# Autodesk Inventor assembly: assembly
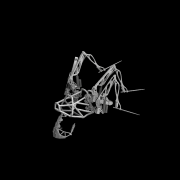
[picture p0: Inventor's stored thumbnail of the model, 180x180]
Saved by Autodesk Inventor 2020 (Build 240168000, 168)
## iProperties
Created: 2020-03-24
Part Number: assembly
Document SubType Name: Assembly
Designer: valer
Author: valer
## Documents named in this file (30)
- C:\Users\valer\Desktop\drummingrobot\src\Robot.iam
- C:\Users\valer\Desktop\drummingrobot\src\Chest.ipt
- C:\Users\valer\Desktop\drummingrobot\src\HeadScaled.ipt
- C:\Users\valer\Desktop\drummingrobot\src\UpperArm.ipt
- C:\Users\valer\Desktop\drummingrobot\src\UpperArmBracket.ipt
- C:\Users\valer\Desktop\drummingrobot\src\external\ShoulderConnectingRod.ipt
- C:\Users\valer\Desktop\drummingrobot\src\Forearm.ipt
- C:\Users\valer\Desktop\drummingrobot\src\external\Drumstick.ipt
- C:\Users\valer\Desktop\drummingrobot\src\external\ForearmShaftCollar.ipt
- C:\Users\valer\Desktop\drummingrobot\src\external\RodEndFixed.ipt
- C:\Users\valer\Desktop\drummingrobot\src\ShoulderBracket.ipt
- C:\Users\valer\Desktop\drummingrobot\src\ChestShoulderBracket.ipt
- C:\Users\valer\Desktop\drummingrobot\src\ChestShoulderBracketMirror.ipt
- C:\Users\valer\Desktop\drummingrobot\src\external\UpperArmActuatorBody.ipt
- C:\Users\valer\Desktop\drummingrobot\src\external\UpperArmActuatorShaft.ipt
- C:\Users\valer\Desktop\drummingrobot\src\external\ForearmActuatorBody.ipt
- C:\Users\valer\Desktop\drummingrobot\src\external\ForearmActuatorShaft.ipt
- C:\Users\valer\Desktop\drummingrobot\src\external\Drums.ipt
- C:\Users\valer\Desktop\drummingrobot\src\ForearmActuatorConnector.ipt
- C:\Users\valer\Desktop\drummingrobot\src\external\ArmRotationServoBody.ipt
- C:\Users\valer\Desktop\drummingrobot\src\external\ArmRotationServoHead.ipt
- C:\Users\valer\Desktop\drummingrobot\src\external\PullSolenoid.ipt
- C:\Users\valer\Desktop\drummingrobot\src\PullSolenoidArmBracket.ipt
- C:\Users\valer\Desktop\drummingrobot\src\UpperShoulderBracket.ipt
- C:\Users\valer\Desktop\drummingrobot\src\UpperArmActuatorBracketAlt.ipt
- C:\Users\valer\Desktop\drummingrobot\src\external\ShockAbsorberDerived.ipt
- C:\Users\valer\Desktop\drummingrobot\src\Spine.ipt
- C:\Users\valer\Desktop\drummingrobot\src\SpineLinkTop.ipt
- C:\Users\valer\Desktop\drummingrobot\src\SpineLinkBottom.ipt
- C:\Users\valer\Desktop\drummingrobot\src\Pelvis.iam
## Components (132 placed, 29 different names)
1. Chest:1 — Angle:6, Mate:117, Mate:118, Mate:119, Mate:120, Mate:121, Mate:122, Mate:130, Mate:131, Mate:132, Mate:133, Mate:134, Mate:157, Angle:12, Mate:425, Mate:426, Mate:427, Mate:428, Mate:429, Mate:430, Mate:431, Mate:432, Mate:433, Mate:434, Mate:435, Mate:436, Angle:18, Mate:568, Mate:571, Angle:23
2. HeadScaled:1 — Angle:6
3. Drumstick:1 — Mate:79, Flush:23, Mate:424
4. ShaftCollar1/2:1 — Mate:79, Mate:290, Mate:291, Flush:23
5. ChestShoulderBracket:1 — Mate:120, Mate:121, Mate:122, Mate:377, Mate:378, Mate:379, Mate:380, Flush:31
6. ChestShoulderBracketMirror:1 — Mate:117, Mate:118, Mate:119, Mate:395, Mate:396, Mate:397, Mate:398
7. ChestShoulderBracket:2 — Mate:130, Mate:131, Mate:157, Mate:160, Mate:162, Mate:213, Mate:214, Flush:28
8. ChestShoulderBracketMirror:2 — Mate:132, Mate:133, Mate:134, Mate:141, Mate:146, Mate:148, Mate:149
9. ChestConnectingRod:5
10. ChestConnectingRod:6
11. RodEnd1/4-1/4-1:9 — Mate:342
12. RodEnd1/4-1/4-1:10 — Mate:148, Mate:149
13. RodEnd1/4-1/4-1:11 — Mate:341
14. RodEnd1/4-1/4-1:12 — Mate:141, Mate:146
15. ChestConnectingRod:7
16. ChestConnectingRod:8
17. RodEnd1/4-1/4-1:13 — Mate:340
18. RodEnd1/4-1/4-1:14 — Mate:162, Mate:214
19. RodEnd1/4-1/4-1:15 — Mate:339
20. RodEnd1/4-1/4-1:16 — Mate:160, Mate:213
21. UpperArmActuatorBody:1 — Mate:182, Mate:183, Mate:423
22. Forearm:1 — Flush:17, Mate:227, Mate:239, Mate:244, Mate:290, Mate:291, Mate:293, Mate:296
23. UpperArmActuatorShaft:2 — Mate:182, Mate:183, Mate:238, Flush:20
24. ForearmActuatorBody:1 — Mate:231, Mate:232, Mate:234, Flush:19
25. Drums:1
26. ForearmActuatorShaft:3 — Flush:17, Mate:231, Mate:232, Mate:241, Mate:243, Angle:10, Mate:246
27. UpperArm:3 — Mate:227, Mate:234, Mate:238, Flush:19, Flush:20, Mate:249, Mate:287
28. ForearmActuatorConnector:1 — Mate:239, Mate:241, Mate:245, Angle:10, Mate:246
29. ForearmActuatorConnector:2 — Mate:243, Mate:244, Mate:245
30. UpperArmBracket:5 — Mate:249, Mate:287, Mate:420, Mate:421, Mate:454
31. ArmRotationServoBody:1 — Mate:258, Mate:259, Angle:12, Mate:384, Mate:386, Mate:387, Mate:388, Mate:402
32. ArmRotationServoHead:1 — Mate:258, Mate:259, Mate:417, Mate:418, Mate:453
33. PullSolenoid:1 — Mate:294, Mate:295, Angle:16, Mate:424
34. PullSolenoidArmBracket:1 — Mate:293, Mate:294, Mate:295, Mate:296, Angle:16
35. Forearm:2 — Mate:343, Mate:347, Mate:352, Mate:353
36. ShaftCollar1/2:2 — Mate:354, Flush:29
37. ShoulderBracket:6 — Mate:332, Mate:333, Flush:28, Mate:339, Mate:340, Mate:403
38. UpperArmActuatorBody:2 — Mate:416
39. UpperArmActuatorShaft:3
40. ForearmActuatorBody:2
41. ForearmActuatorShaft:4 — Mate:349, Mate:350, Mate:351, Angle:13
42. UpperArm:4
43. UpperArmBracket:6 — Mate:413, Mate:414, Mate:415
44. ArmRotationServoBody:2 — Mate:330, Mate:331, Mate:332, Mate:333, Mate:334, Mate:335, Mate:403, Mate:404
45. ShoulderBracket:7 — Mate:334, Mate:335, Mate:341, Mate:342, Mate:404
46. PullSolenoid:2 — Mate:344, Mate:345, Angle:14, Mate:355
47. PullSolenoidArmBracket:2 — Mate:343, Mate:344, Mate:345, Mate:347, Angle:14
48. ArmRotationServoHead:2 — Mate:330, Mate:331, Mate:410, Mate:411, Mate:412
49. ForearmActuatorConnector:3 — Mate:349, Mate:351, Mate:353
50. ForearmActuatorConnector:4 — Mate:350, Mate:352, Angle:13
51. Drumstick:2 — Mate:354, Mate:355, Flush:29
52. UpperShoulderBracket:1 — Mate:384, Flush:31, Mate:388, Mate:389, Mate:390
53. UpperShoulderBracket:2 — Mate:386, Mate:387, Mate:391, Mate:392, Mate:401, Mate:402
54. RodEnd1/4-1/4-1:17 — Mate:382, Mate:389
55. RodEnd1/4-1/4-1:18 — Mate:381, Mate:390, Mate:406
56. RodEnd1/4-1/4-1:19 — Mate:377, Mate:378, Mate:382, Mate:405
57. RodEnd1/4-1/4-1:20 — Mate:379, Mate:380, Mate:381
58. RodEnd1/4-1/4-1:21 — Mate:392, Mate:400, Mate:408
59. RodEnd1/4-1/4-1:22 — Mate:391, Mate:399, Mate:401, Mate:407
60. RodEnd1/4-1/4-1:23 — Mate:395, Mate:398, Mate:399
61. RodEnd1/4-1/4-1:24 — Mate:396, Mate:397, Mate:400, Mate:573
62. ChestConnectingRod:9 — Mate:405
63. ChestConnectingRod:10 — Mate:406
64. ChestConnectingRod:11 — Mate:407
65. ChestConnectingRod:12 — Mate:408
66. UpperArmActuatorBracketAlt:1 — Mate:410, Mate:411, Mate:412, Mate:413, Mate:414, Mate:415, Mate:416
67. UpperArmActuatorBracketAlt:2 — Mate:417, Mate:418, Mate:420, Mate:421, Mate:423, Mate:453, Mate:454
68. ChestShoulderBracket:3 — Mate:428, Mate:429, Mate:430, Mate:437, Mate:438, Mate:439, Mate:440
69. ChestShoulderBracketMirror:3 — Mate:425, Mate:426, Mate:427, Mate:441, Mate:442, Mate:443, Mate:444, Mate:570
70. ChestShoulderBracket:4 — Mate:431, Mate:432, Mate:433, Mate:445, Mate:446, Mate:447, Mate:448
71. ChestShoulderBracketMirror:4 — Mate:434, Mate:435, Mate:436, Mate:449, Mate:451, Mate:452
72. RodEnd1/4-1/4-1:25 — Mate:439, Mate:440
73. RodEnd1/4-1/4-1:26 — Mate:437, Mate:438, Mate:481
74. RodEnd1/4-1/4-1:27 — Mate:442, Mate:444, Mate:480
75. RodEnd1/4-1/4-1:28 — Mate:441, Mate:443, Mate:479
76. RodEnd1/4-1/4-1:29 — Mate:447, Mate:448, Mate:499
77. RodEnd1/4-1/4-1:30 — Mate:445, Mate:446, Mate:498
78. RodEnd1/4-1/4-1:31 — Mate:452, Mate:497
79. RodEnd1/4-1/4-1:32 — Mate:449, Mate:451, Mate:496
80. ArmRotationServoBody:3 — Mate:469
81. ArmRotationServoHead:3 — Mate:509, Mate:510, Mate:511
82. UpperShoulderBracket:3 — Mate:469, Mate:474, Mate:476, Mate:567
83. UpperShoulderBracket:4 — Mate:471
84. ArmRotationServoBody:4 — Mate:482, Mate:483, Mate:484, Mate:485, Mate:486, Mate:487, Angle:18
85. ArmRotationServoHead:4 — Mate:521, Mate:522, Mate:523
86. RodEnd1/4-1/4-1:33 — Mate:471, Mate:479
87. RodEnd1/4-1/4-1:34 — Mate:480
88. RodEnd1/4-1/4-1:35 — Mate:481
89. RodEnd1/4-1/4-1:36 — Mate:474, Mate:476
90. RodEnd1/4-1/4-1:37 — Mate:492, Mate:494, Mate:498
91. RodEnd1/4-1/4-1:38 — Mate:493, Mate:495, Mate:499
92. RodEnd1/4-1/4-1:39 — Mate:489, Mate:491, Mate:497
93. RodEnd1/4-1/4-1:40 — Mate:496
94. ShoulderBracket:8 — Mate:482, Mate:483, Mate:484, Mate:489, Mate:491
95. ShoulderBracket:9 — Mate:485, Mate:486, Mate:487, Mate:492, Mate:493, Mate:494, Mate:495, Mate:566
96. UpperArmActuatorBody:3
97. UpperArmActuatorShaft:4
98. UpperArm:5 — Mate:558, Mate:559, Mate:560
99. UpperArmBracket:7
100. UpperArmActuatorBracketAlt:3 — Mate:509, Mate:510, Mate:511
101. UpperArmActuatorBody:4
102. UpperArmActuatorShaft:5
103. UpperArm:6 — Mate:561, Mate:562, Mate:563
104. UpperArmBracket:8
105. UpperArmActuatorBracketAlt:4 — Mate:521, Mate:522, Mate:523
106. Forearm:3 — Mate:558, Mate:559
107. Drumstick:3 — Mate:556
108. ShaftCollar1/2:3 — Mate:556
109. ForearmActuatorBody:3 — Mate:560
110. ForearmActuatorShaft:5
111. ForearmActuatorConnector:5
112. ForearmActuatorConnector:6
113. PullSolenoid:3
114. PullSolenoidArmBracket:3
115. Forearm:4 — Mate:561, Mate:562
116. Drumstick:4 — Mate:557, Mate:564
117. ShaftCollar1/2:4 — Mate:557
118. ForearmActuatorBody:4 — Mate:563
119. ForearmActuatorShaft:6
120. ForearmActuatorConnector:7
121. ForearmActuatorConnector:8
122. PullSolenoid:4 — Mate:564
123. PullSolenoidArmBracket:4
124. ShockAbsorberDerived:1 — Mate:566, Mate:570
125. ShockAbsorberDerived:2 — Mate:567, Mate:568
126. ShockAbsorberDerived:3 — Mate:573
127. ShockAbsorberDerived:4 — Mate:571
128. ShockAbsorberDerived:5 — Mate:585, Mate:586
129. Spine:1 — Mate:574, Mate:575, Mate:576, Mate:579, Mate:580, Mate:581, Mate:582, Mate:583, Mate:584, Angle:23
130. SpineLinkTop:1 — Mate:574, Mate:575, Mate:576
131. SpineLinkBottom:1 — Mate:579, Mate:580, Mate:581
132. Pelvis:1 [sub-assembly] — Mate:582, Mate:583, Mate:584, Mate:585, Mate:586
## Relationships (294: Mate 266, Flush 16, Angle 12)
- Angle:6 (0 deg): Chest:1 ↔ HeadScaled:1
- Mate:79: Drumstick:1 ↔ ShaftCollar1/2:1
- Mate:117: Chest:1 ↔ ChestShoulderBracketMirror:1
- Mate:118: Chest:1 ↔ ChestShoulderBracketMirror:1
- Mate:119: Chest:1 ↔ ChestShoulderBracketMirror:1
- Mate:120: Chest:1 ↔ ChestShoulderBracket:1
- Mate:121: Chest:1 ↔ ChestShoulderBracket:1
- Mate:122: Chest:1 ↔ ChestShoulderBracket:1
- Mate:130: Chest:1 ↔ ChestShoulderBracket:2
- Mate:131: Chest:1 ↔ ChestShoulderBracket:2
- Mate:132: Chest:1 ↔ ChestShoulderBracketMirror:2
- Mate:133: Chest:1 ↔ ChestShoulderBracketMirror:2
- Mate:134: Chest:1 ↔ ChestShoulderBracketMirror:2
- [Mate]: ChestConnectingRod:6 ↔ RodEnd1/4-1/4-1:9
- [Mate]: ChestConnectingRod:6 ↔ RodEnd1/4-1/4-1:10
- [Mate]: ChestConnectingRod:5 ↔ RodEnd1/4-1/4-1:11
- [Mate]: ChestConnectingRod:5 ↔ RodEnd1/4-1/4-1:12
- [Mate] (-25.4 mm): ChestConnectingRod:6 ↔ RodEnd1/4-1/4-1:10
- [Mate] (-25.4 mm): ChestConnectingRod:5 ↔ RodEnd1/4-1/4-1:12
- Mate:141: ChestShoulderBracketMirror:2 ↔ RodEnd1/4-1/4-1:12
- Mate:146: ChestShoulderBracketMirror:2 ↔ RodEnd1/4-1/4-1:12
- Mate:148: ChestShoulderBracketMirror:2 ↔ RodEnd1/4-1/4-1:10
- Mate:149: ChestShoulderBracketMirror:2 ↔ RodEnd1/4-1/4-1:10
- [Mate]: ChestConnectingRod:8 ↔ RodEnd1/4-1/4-1:13
- [Mate]: ChestConnectingRod:8 ↔ RodEnd1/4-1/4-1:14
- [Mate]: ChestConnectingRod:7 ↔ RodEnd1/4-1/4-1:15
- [Mate]: ChestConnectingRod:7 ↔ RodEnd1/4-1/4-1:16
- [Mate] (-25.4 mm): ChestConnectingRod:8 ↔ RodEnd1/4-1/4-1:14
- [Mate] (-25.4 mm): ChestConnectingRod:7 ↔ RodEnd1/4-1/4-1:16
- Mate:157: Chest:1 ↔ ChestShoulderBracket:2
- Mate:160: ChestShoulderBracket:2 ↔ RodEnd1/4-1/4-1:16
- Mate:162: ChestShoulderBracket:2 ↔ RodEnd1/4-1/4-1:14
- Mate:182: UpperArmActuatorBody:1 ↔ UpperArmActuatorShaft:2
- Mate:183: UpperArmActuatorBody:1 ↔ UpperArmActuatorShaft:2
- Mate:213: ChestShoulderBracket:2 ↔ RodEnd1/4-1/4-1:16
- Mate:214: ChestShoulderBracket:2 ↔ RodEnd1/4-1/4-1:14
- Flush:17: Forearm:1 ↔ ForearmActuatorShaft:3
- Mate:227: Forearm:1 ↔ UpperArm:3
- Mate:231: ForearmActuatorBody:1 ↔ ForearmActuatorShaft:3
- Mate:232: ForearmActuatorBody:1 ↔ ForearmActuatorShaft:3
- Mate:234: ForearmActuatorBody:1 ↔ UpperArm:3
- Mate:238: UpperArmActuatorShaft:2 ↔ UpperArm:3
- Flush:19: ForearmActuatorBody:1 ↔ UpperArm:3
- Flush:20: UpperArmActuatorShaft:2 ↔ UpperArm:3
- Mate:239: Forearm:1 ↔ ForearmActuatorConnector:1
- Mate:241: ForearmActuatorShaft:3 ↔ ForearmActuatorConnector:1
- Mate:243: ForearmActuatorShaft:3 ↔ ForearmActuatorConnector:2
- Mate:244: Forearm:1 ↔ ForearmActuatorConnector:2
- Mate:245: ForearmActuatorConnector:1 ↔ ForearmActuatorConnector:2
- Angle:10 (-180 deg): ForearmActuatorShaft:3 ↔ ForearmActuatorConnector:1
- Mate:246: ForearmActuatorShaft:3 ↔ ForearmActuatorConnector:1
- Mate:249: UpperArm:3 ↔ UpperArmBracket:5
- Mate:258: ArmRotationServoBody:1 ↔ ArmRotationServoHead:1
- Mate:259: ArmRotationServoBody:1 ↔ ArmRotationServoHead:1
- Angle:12 (0 deg): Chest:1 ↔ ArmRotationServoBody:1
- Mate:287: UpperArm:3 ↔ UpperArmBracket:5
- Mate:290: ShaftCollar1/2:1 ↔ Forearm:1
- Mate:291 (8.4667 mm): ShaftCollar1/2:1 ↔ Forearm:1
- Mate:293: Forearm:1 ↔ PullSolenoidArmBracket:1
- Mate:294: PullSolenoid:1 ↔ PullSolenoidArmBracket:1
- Mate:295: PullSolenoid:1 ↔ PullSolenoidArmBracket:1
- Mate:296: Forearm:1 ↔ PullSolenoidArmBracket:1
- Flush:23 (302.5394 mm): Drumstick:1 ↔ ShaftCollar1/2:1
- [Mate]: UpperArmActuatorBody:2 ↔ UpperArmActuatorShaft:3
- [Mate]: UpperArmActuatorBody:2 ↔ UpperArmActuatorShaft:3
- [Flush]: Forearm:2 ↔ ForearmActuatorShaft:4
- [Mate]: Forearm:2 ↔ UpperArm:4
- [Mate]: ForearmActuatorBody:2 ↔ ForearmActuatorShaft:4
- [Mate]: ForearmActuatorBody:2 ↔ ForearmActuatorShaft:4
- [Mate]: ForearmActuatorBody:2 ↔ UpperArm:4
- [Mate]: UpperArmActuatorShaft:3 ↔ UpperArm:4
- [Flush]: ForearmActuatorBody:2 ↔ UpperArm:4
- [Flush]: UpperArmActuatorShaft:3 ↔ UpperArm:4
- [Mate]: UpperArm:4 ↔ UpperArmBracket:6
- [Mate]: UpperArm:4 ↔ UpperArmBracket:6
- [Mate]: Forearm:2 ↔ ShaftCollar1/2:2
- [Mate] (8.4667 mm): Forearm:2 ↔ ShaftCollar1/2:2
- Mate:330: ArmRotationServoBody:2 ↔ ArmRotationServoHead:2
- Mate:331: ArmRotationServoBody:2 ↔ ArmRotationServoHead:2
- Mate:332: ShoulderBracket:6 ↔ ArmRotationServoBody:2
- Mate:333: ShoulderBracket:6 ↔ ArmRotationServoBody:2
- Mate:334: ArmRotationServoBody:2 ↔ ShoulderBracket:7
- Mate:335: ArmRotationServoBody:2 ↔ ShoulderBracket:7
- Flush:28: ChestShoulderBracket:2 ↔ ShoulderBracket:6
- Mate:339: RodEnd1/4-1/4-1:15 ↔ ShoulderBracket:6
- Mate:340: RodEnd1/4-1/4-1:13 ↔ ShoulderBracket:6
- Mate:341: RodEnd1/4-1/4-1:11 ↔ ShoulderBracket:7
- Mate:342: RodEnd1/4-1/4-1:9 ↔ ShoulderBracket:7
- Mate:343: Forearm:2 ↔ PullSolenoidArmBracket:2
- Mate:344: PullSolenoid:2 ↔ PullSolenoidArmBracket:2
- Mate:345: PullSolenoid:2 ↔ PullSolenoidArmBracket:2
- Mate:347: Forearm:2 ↔ PullSolenoidArmBracket:2
- [Mate]: ForearmActuatorConnector:3 ↔ ForearmActuatorConnector:4
- Mate:349: ForearmActuatorShaft:4 ↔ ForearmActuatorConnector:3
- Mate:350: ForearmActuatorShaft:4 ↔ ForearmActuatorConnector:4
- Mate:351: ForearmActuatorShaft:4 ↔ ForearmActuatorConnector:3
- Mate:352: Forearm:2 ↔ ForearmActuatorConnector:4
- Mate:353: Forearm:2 ↔ ForearmActuatorConnector:3
- Angle:13 (6.23 deg): ForearmActuatorShaft:4 ↔ ForearmActuatorConnector:4
- Angle:14 (0 deg): PullSolenoid:2 ↔ PullSolenoidArmBracket:2
- Mate:354: ShaftCollar1/2:2 ↔ Drumstick:2
- Mate:355: PullSolenoid:2 ↔ Drumstick:2
- Flush:29 (107.2642 mm): ShaftCollar1/2:2 ↔ Drumstick:2
- Mate:377: ChestShoulderBracket:1 ↔ RodEnd1/4-1/4-1:19
- Mate:378: ChestShoulderBracket:1 ↔ RodEnd1/4-1/4-1:19
- Mate:379: ChestShoulderBracket:1 ↔ RodEnd1/4-1/4-1:20
- Mate:380: ChestShoulderBracket:1 ↔ RodEnd1/4-1/4-1:20
- Mate:381: RodEnd1/4-1/4-1:18 ↔ RodEnd1/4-1/4-1:20
- Mate:382: RodEnd1/4-1/4-1:17 ↔ RodEnd1/4-1/4-1:19
- Mate:384: ArmRotationServoBody:1 ↔ UpperShoulderBracket:1
- Flush:31: ChestShoulderBracket:1 ↔ UpperShoulderBracket:1
- Mate:386: ArmRotationServoBody:1 ↔ UpperShoulderBracket:2
- Mate:387: ArmRotationServoBody:1 ↔ UpperShoulderBracket:2
- Mate:388: ArmRotationServoBody:1 ↔ UpperShoulderBracket:1
- Mate:389: UpperShoulderBracket:1 ↔ RodEnd1/4-1/4-1:17
- Mate:390: UpperShoulderBracket:1 ↔ RodEnd1/4-1/4-1:18
- Mate:391: UpperShoulderBracket:2 ↔ RodEnd1/4-1/4-1:22
- Mate:392: UpperShoulderBracket:2 ↔ RodEnd1/4-1/4-1:21
- Mate:395: ChestShoulderBracketMirror:1 ↔ RodEnd1/4-1/4-1:23
- Mate:396: ChestShoulderBracketMirror:1 ↔ RodEnd1/4-1/4-1:24
- Mate:397: ChestShoulderBracketMirror:1 ↔ RodEnd1/4-1/4-1:24
- Mate:398: ChestShoulderBracketMirror:1 ↔ RodEnd1/4-1/4-1:23
- Mate:399: RodEnd1/4-1/4-1:22 ↔ RodEnd1/4-1/4-1:23
- Mate:400: RodEnd1/4-1/4-1:21 ↔ RodEnd1/4-1/4-1:24
- Mate:401: UpperShoulderBracket:2 ↔ RodEnd1/4-1/4-1:22
- Mate:402: ArmRotationServoBody:1 ↔ UpperShoulderBracket:2
- Mate:403: ShoulderBracket:6 ↔ ArmRotationServoBody:2
- Mate:404: ArmRotationServoBody:2 ↔ ShoulderBracket:7
- Mate:405: RodEnd1/4-1/4-1:19 ↔ ChestConnectingRod:9
- Mate:406: RodEnd1/4-1/4-1:18 ↔ ChestConnectingRod:10
- Mate:407: RodEnd1/4-1/4-1:22 ↔ ChestConnectingRod:11
- Mate:408: RodEnd1/4-1/4-1:21 ↔ ChestConnectingRod:12
- Mate:410: ArmRotationServoHead:2 ↔ UpperArmActuatorBracketAlt:1
- Mate:411: ArmRotationServoHead:2 ↔ UpperArmActuatorBracketAlt:1
- Mate:412: ArmRotationServoHead:2 ↔ UpperArmActuatorBracketAlt:1
- Mate:413: UpperArmBracket:6 ↔ UpperArmActuatorBracketAlt:1
- Mate:414: UpperArmBracket:6 ↔ UpperArmActuatorBracketAlt:1
- Mate:415: UpperArmBracket:6 ↔ UpperArmActuatorBracketAlt:1
- Mate:416: UpperArmActuatorBody:2 ↔ UpperArmActuatorBracketAlt:1
- Mate:417: ArmRotationServoHead:1 ↔ UpperArmActuatorBracketAlt:2
- Mate:418: ArmRotationServoHead:1 ↔ UpperArmActuatorBracketAlt:2
- Mate:420: UpperArmBracket:5 ↔ UpperArmActuatorBracketAlt:2
- Mate:421: UpperArmBracket:5 ↔ UpperArmActuatorBracketAlt:2
- Mate:423: UpperArmActuatorBody:1 ↔ UpperArmActuatorBracketAlt:2
- Angle:16 (180 deg): PullSolenoid:1 ↔ PullSolenoidArmBracket:1
- Mate:424: Drumstick:1 ↔ PullSolenoid:1
- Mate:425: Chest:1 ↔ ChestShoulderBracketMirror:3
- Mate:426: Chest:1 ↔ ChestShoulderBracketMirror:3
- Mate:427: Chest:1 ↔ ChestShoulderBracketMirror:3
- Mate:428: Chest:1 ↔ ChestShoulderBracket:3
- Mate:429: Chest:1 ↔ ChestShoulderBracket:3
- Mate:430: Chest:1 ↔ ChestShoulderBracket:3
- Mate:431: Chest:1 ↔ ChestShoulderBracket:4
- Mate:432: Chest:1 ↔ ChestShoulderBracket:4
- Mate:433: Chest:1 ↔ ChestShoulderBracket:4
- Mate:434: Chest:1 ↔ ChestShoulderBracketMirror:4
- Mate:435: Chest:1 ↔ ChestShoulderBracketMirror:4
- Mate:436: Chest:1 ↔ ChestShoulderBracketMirror:4
- Mate:437: ChestShoulderBracket:3 ↔ RodEnd1/4-1/4-1:26
- Mate:438: ChestShoulderBracket:3 ↔ RodEnd1/4-1/4-1:26
- Mate:439: ChestShoulderBracket:3 ↔ RodEnd1/4-1/4-1:25
- Mate:440: ChestShoulderBracket:3 ↔ RodEnd1/4-1/4-1:25
- Mate:441: ChestShoulderBracketMirror:3 ↔ RodEnd1/4-1/4-1:28
- Mate:442: ChestShoulderBracketMirror:3 ↔ RodEnd1/4-1/4-1:27
- Mate:443: ChestShoulderBracketMirror:3 ↔ RodEnd1/4-1/4-1:28
- Mate:444: ChestShoulderBracketMirror:3 ↔ RodEnd1/4-1/4-1:27
- Mate:445: ChestShoulderBracket:4 ↔ RodEnd1/4-1/4-1:30
- Mate:446: ChestShoulderBracket:4 ↔ RodEnd1/4-1/4-1:30
- Mate:447: ChestShoulderBracket:4 ↔ RodEnd1/4-1/4-1:29
- Mate:448: ChestShoulderBracket:4 ↔ RodEnd1/4-1/4-1:29
- Mate:449: ChestShoulderBracketMirror:4 ↔ RodEnd1/4-1/4-1:32
- Mate:451: ChestShoulderBracketMirror:4 ↔ RodEnd1/4-1/4-1:32
- Mate:452: ChestShoulderBracketMirror:4 ↔ RodEnd1/4-1/4-1:31
- Mate:453: ArmRotationServoHead:1 ↔ UpperArmActuatorBracketAlt:2
- Mate:454: UpperArmBracket:5 ↔ UpperArmActuatorBracketAlt:2
- [Mate]: ArmRotationServoBody:3 ↔ UpperShoulderBracket:3
- [Mate]: ArmRotationServoBody:3 ↔ UpperShoulderBracket:4
- [Mate]: ArmRotationServoBody:3 ↔ UpperShoulderBracket:4
- [Mate]: ArmRotationServoBody:3 ↔ UpperShoulderBracket:3
- [Mate]: ArmRotationServoBody:3 ↔ UpperShoulderBracket:4
- [Mate]: ArmRotationServoBody:4 ↔ ArmRotationServoHead:4
- [Mate]: ArmRotationServoBody:4 ↔ ArmRotationServoHead:4
- Mate:469: ArmRotationServoBody:3 ↔ UpperShoulderBracket:3
- Mate:471: UpperShoulderBracket:4 ↔ RodEnd1/4-1/4-1:33
- Mate:474: UpperShoulderBracket:3 ↔ RodEnd1/4-1/4-1:36
- Mate:476: UpperShoulderBracket:3 ↔ RodEnd1/4-1/4-1:36
- Mate:479: RodEnd1/4-1/4-1:28 ↔ RodEnd1/4-1/4-1:33
- Mate:480: RodEnd1/4-1/4-1:27 ↔ RodEnd1/4-1/4-1:34
- Mate:481: RodEnd1/4-1/4-1:26 ↔ RodEnd1/4-1/4-1:35
- Mate:482: ArmRotationServoBody:4 ↔ ShoulderBracket:8
- Mate:483: ArmRotationServoBody:4 ↔ ShoulderBracket:8
- Mate:484: ArmRotationServoBody:4 ↔ ShoulderBracket:8
- Mate:485: ArmRotationServoBody:4 ↔ ShoulderBracket:9
- Mate:486: ArmRotationServoBody:4 ↔ ShoulderBracket:9
- Mate:487: ArmRotationServoBody:4 ↔ ShoulderBracket:9
- Angle:18 (0 deg): Chest:1 ↔ ArmRotationServoBody:4
- Mate:489: RodEnd1/4-1/4-1:39 ↔ ShoulderBracket:8
- Mate:491: RodEnd1/4-1/4-1:39 ↔ ShoulderBracket:8
- Mate:492: RodEnd1/4-1/4-1:37 ↔ ShoulderBracket:9
- Mate:493: RodEnd1/4-1/4-1:38 ↔ ShoulderBracket:9
- Mate:494: RodEnd1/4-1/4-1:37 ↔ ShoulderBracket:9
- Mate:495: RodEnd1/4-1/4-1:38 ↔ ShoulderBracket:9
- Mate:496: RodEnd1/4-1/4-1:32 ↔ RodEnd1/4-1/4-1:40
- Mate:497: RodEnd1/4-1/4-1:31 ↔ RodEnd1/4-1/4-1:39
- Mate:498: RodEnd1/4-1/4-1:30 ↔ RodEnd1/4-1/4-1:37
- Mate:499: RodEnd1/4-1/4-1:29 ↔ RodEnd1/4-1/4-1:38
- [Mate]: UpperArmActuatorBody:3 ↔ UpperArmActuatorShaft:4
- [Mate]: UpperArmActuatorBody:3 ↔ UpperArmActuatorShaft:4
- [Mate]: UpperArmActuatorShaft:4 ↔ UpperArm:5
- [Flush]: UpperArmActuatorShaft:4 ↔ UpperArm:5
- [Mate]: UpperArm:5 ↔ UpperArmBracket:7
- [Mate]: UpperArm:5 ↔ UpperArmBracket:7
- [Mate]: UpperArmBracket:7 ↔ UpperArmActuatorBracketAlt:3
- [Mate]: UpperArmBracket:7 ↔ UpperArmActuatorBracketAlt:3
- [Mate]: UpperArmBracket:7 ↔ UpperArmActuatorBracketAlt:3
- [Mate]: UpperArmActuatorBody:3 ↔ UpperArmActuatorBracketAlt:3
- Mate:509: ArmRotationServoHead:3 ↔ UpperArmActuatorBracketAlt:3
- Mate:510: ArmRotationServoHead:3 ↔ UpperArmActuatorBracketAlt:3
- Mate:511: ArmRotationServoHead:3 ↔ UpperArmActuatorBracketAlt:3
- [Mate]: UpperArmActuatorBody:4 ↔ UpperArmActuatorShaft:5
- [Mate]: UpperArmActuatorBody:4 ↔ UpperArmActuatorShaft:5
- [Mate]: UpperArmActuatorShaft:5 ↔ UpperArm:6
- [Flush]: UpperArmActuatorShaft:5 ↔ UpperArm:6
- [Mate]: UpperArm:6 ↔ UpperArmBracket:8
- [Mate]: UpperArm:6 ↔ UpperArmBracket:8
- [Mate]: UpperArmBracket:8 ↔ UpperArmActuatorBracketAlt:4
- [Mate]: UpperArmBracket:8 ↔ UpperArmActuatorBracketAlt:4
- [Mate]: UpperArmBracket:8 ↔ UpperArmActuatorBracketAlt:4
- [Mate]: UpperArmActuatorBody:4 ↔ UpperArmActuatorBracketAlt:4
- Mate:521: ArmRotationServoHead:4 ↔ UpperArmActuatorBracketAlt:4
- Mate:522: ArmRotationServoHead:4 ↔ UpperArmActuatorBracketAlt:4
- Mate:523: ArmRotationServoHead:4 ↔ UpperArmActuatorBracketAlt:4
- [Flush]: Forearm:3 ↔ ForearmActuatorShaft:5
- [Mate]: ForearmActuatorBody:3 ↔ ForearmActuatorShaft:5
- [Mate]: Forearm:3 ↔ ForearmActuatorConnector:5
- [Mate]: ForearmActuatorShaft:5 ↔ ForearmActuatorConnector:5
- [Mate]: ForearmActuatorShaft:5 ↔ ForearmActuatorConnector:6
- [Mate]: Forearm:3 ↔ ForearmActuatorConnector:6
- [Mate]: ForearmActuatorConnector:5 ↔ ForearmActuatorConnector:6
- [Angle] (-180 deg): ForearmActuatorShaft:5 ↔ ForearmActuatorConnector:5
- [Mate]: ForearmActuatorShaft:5 ↔ ForearmActuatorConnector:5
- [Mate]: Forearm:3 ↔ ShaftCollar1/2:3
- [Mate] (8.4667 mm): Forearm:3 ↔ ShaftCollar1/2:3
- [Mate]: Forearm:3 ↔ PullSolenoidArmBracket:3
- [Mate]: PullSolenoid:3 ↔ PullSolenoidArmBracket:3
- [Mate]: PullSolenoid:3 ↔ PullSolenoidArmBracket:3
- [Mate]: Forearm:3 ↔ PullSolenoidArmBracket:3
- [Flush] (302.5394 mm): Drumstick:3 ↔ ShaftCollar1/2:3
- [Angle] (180 deg): PullSolenoid:3 ↔ PullSolenoidArmBracket:3
- [Mate]: Drumstick:3 ↔ PullSolenoid:3
- [Flush]: Forearm:4 ↔ ForearmActuatorShaft:6
- [Mate]: ForearmActuatorBody:4 ↔ ForearmActuatorShaft:6
- [Mate]: Forearm:4 ↔ ForearmActuatorConnector:7
- [Mate]: ForearmActuatorShaft:6 ↔ ForearmActuatorConnector:7
- [Mate]: ForearmActuatorShaft:6 ↔ ForearmActuatorConnector:8
- [Mate]: Forearm:4 ↔ ForearmActuatorConnector:8
- [Mate]: ForearmActuatorConnector:7 ↔ ForearmActuatorConnector:8
- [Angle] (-180 deg): ForearmActuatorShaft:6 ↔ ForearmActuatorConnector:7
- [Mate]: ForearmActuatorShaft:6 ↔ ForearmActuatorConnector:7
- [Mate]: Forearm:4 ↔ ShaftCollar1/2:4
- [Mate] (8.4667 mm): Forearm:4 ↔ ShaftCollar1/2:4
- [Mate]: Forearm:4 ↔ PullSolenoidArmBracket:4
- [Mate]: PullSolenoid:4 ↔ PullSolenoidArmBracket:4
- [Mate]: PullSolenoid:4 ↔ PullSolenoidArmBracket:4
- [Mate]: Forearm:4 ↔ PullSolenoidArmBracket:4
- [Flush] (302.5394 mm): Drumstick:4 ↔ ShaftCollar1/2:4
- [Angle] (180 deg): PullSolenoid:4 ↔ PullSolenoidArmBracket:4
- Mate:556: Drumstick:3 ↔ ShaftCollar1/2:3
- Mate:557: Drumstick:4 ↔ ShaftCollar1/2:4
- Mate:558: UpperArm:5 ↔ Forearm:3
- Mate:559: UpperArm:5 ↔ Forearm:3
- Mate:560: UpperArm:5 ↔ ForearmActuatorBody:3
- Mate:561: UpperArm:6 ↔ Forearm:4
- Mate:562: UpperArm:6 ↔ Forearm:4
- Mate:563: UpperArm:6 ↔ ForearmActuatorBody:4
- Mate:564: Drumstick:4 ↔ PullSolenoid:4
- Mate:566: ShoulderBracket:9 ↔ ShockAbsorberDerived:1
- Mate:567: UpperShoulderBracket:3 ↔ ShockAbsorberDerived:2
- Mate:568: Chest:1 ↔ ShockAbsorberDerived:2
- Mate:570: ChestShoulderBracketMirror:3 ↔ ShockAbsorberDerived:1
- Mate:571: Chest:1 ↔ ShockAbsorberDerived:4
- Mate:573: RodEnd1/4-1/4-1:24 ↔ ShockAbsorberDerived:3
- Mate:574: Spine:1 ↔ SpineLinkTop:1
- Mate:575: Spine:1 ↔ SpineLinkTop:1
- Mate:576: Spine:1 ↔ SpineLinkTop:1
- Mate:579: Spine:1 ↔ SpineLinkBottom:1
- Mate:580: Spine:1 ↔ SpineLinkBottom:1
- Mate:581: Spine:1 ↔ SpineLinkBottom:1
- Mate:582: Spine:1 ↔ Pelvis:1
- Mate:583: Spine:1 ↔ Pelvis:1
- Mate:584: Spine:1 ↔ Pelvis:1
- Mate:585: ShockAbsorberDerived:5 ↔ Pelvis:1
- Mate:586: ShockAbsorberDerived:5 ↔ Pelvis:1
- Angle:23 (0 deg): Chest:1 ↔ Spine:1
## Named parameters: d244_d149 = 0 mm, d245_d150 = 0 mm, d246_d151 = 0 mm, d247_d152 = 0 mm, d248_d197 = -25.4 mm, d249_d198 = -25.4 mm, d259_d145 = 0 mm, d260_d146 = 0 mm, d261_d147 = 0 mm, d262_d148 = 0 mm, d263_d190 = -25.4 mm, d264_d191 = -25.4 mm, d544_d521 = 0 mm, d547_d529 = 0 mm, d548_d530 = 8.46667 mm, d552_d396 = 0 mm, d553_d397 = 0 mm, d554_d398 = -50.8 mm, d555_d400 = 0 mm, d556_d405 = 0 mm, d557_d409 = 0 mm, d558_d410 = 0 mm, d563_d444 = 0 mm, d565_d384 = 0 mm, d566_d389 = 0 mm, d567_d395 = 0 mm, d568_d294 = 0 mm, d569_d295 = 0 mm, d570_d296 = 0 mm, d571_d297 = -69.85 mm, d600_d423 = 0 mm, d721_d649 = 0 mm, d722_d650 = 0 mm, d723_d667 = 0 mm, d724_d645 = 0 mm, d725_d648 = 0 mm, d733_d454 = 0 mm, d734_d455 = 0 mm, d773_d678 = 0 mm, d774_d679 = 0 mm, d775_d680 = 0 mm, d776_d681 = 0 mm, d777_d544_d521 = 0 mm, d778_d556_d405 = 0 mm, d779_d558_d410 = 0 mm, d780_d563_d444 = 0 mm, d781_d568_d294 = 0 mm, d782_d569_d295 = 0 mm, d783_d570_d296 = 0 mm, d784_d571_d297 = -69.85 mm, d788_d773_d678 = 0 mm, d789_d774_d679 = 0 mm, d790_d775_d680 = 0 mm, d791_d776_d681 = 0 mm, d792_d777_d544_d521 = 0 mm, d793_d778_d556_d405 = 0 mm, d794_d779_d558_d410 = 0 mm, d795_d780_d563_d444 = 0 mm, d796_d781_d568_d294 = 0 mm, d797_d782_d569_d295 = 0 mm, d798_d783_d570_d296 = 0 mm, d799_d784_d571_d297 = -69.85 mm, d803_d689 = 180 deg, d804_d690 = 0 mm, d805_d529 = 0 mm, d806_d530 = 8.46667 mm, d807_d532 = 0 mm, d808_d533 = 0 mm, d809_d534 = 0 mm, d810_d535 = 0 mm, d811_d537 = 302.5394 mm, d812_d384 = 0 mm, d814_d396 = 0 mm, d815_d397 = 0 mm, d816_d398 = -50.8 mm, d817_d417 = 0 mm, d818_d419 = 0 mm, d819_d421 = 0 mm, d820_d422 = 0 mm, d821_d423 = 0 mm, d822_d424 = -180 deg, d823_d425 = 0 mm, d825_d689 = 180 deg, d827_d529 = 0 mm, d828_d530 = 8.46667 mm, d829_d532 = 0 mm, d830_d533 = 0 mm, d831_d534 = 0 mm, d832_d535 = 0 mm, d833_d537 = 302.5394 mm, d834_d384 = 0 mm, d836_d396 = 0 mm, d837_d397 = 0 mm, d838_d398 = -50.8 mm, d839_d417 = 0 mm, d840_d419 = 0 mm, d841_d421 = 0 mm, d842_d422 = 0 mm, d843_d423 = 0 mm, d844_d424 = -180 deg, d845_d425 = 0 mm
